# Autodesk Inventor assembly: Ens. Manija
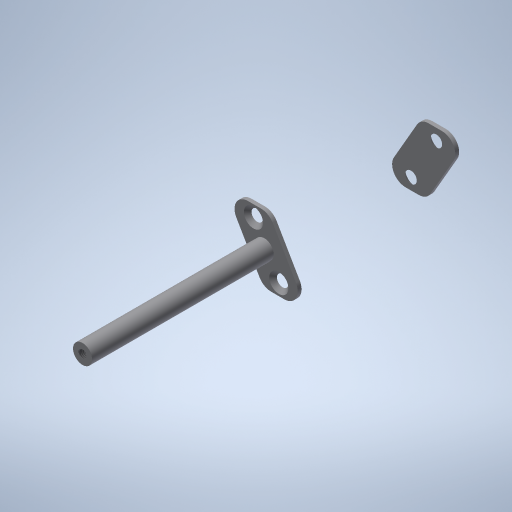
[picture p0: Inventor's stored thumbnail of the model, 512x512]
Saved by Autodesk Inventor 2024.2 (Build 282272000, 272)
## iProperties
Created: 2024-11-25
Part Number: Ens. Manija
Material: Genérico
Document SubType Name: Assembly
Designer: jd.castellanosq
Author: jd.castellanosq
## Documents named in this file (3)
- I:\MICROMECANICA\ALTAS ENERGIAS\Deteccion de Muones\Detectores centelladores\Partes Detectores centelladores\PARTES DC\Manija\Ens. Manija.iam
- I:\MICROMECANICA\ALTAS ENERGIAS\Deteccion de Muones\Detectores centelladores\Partes Detectores centelladores\PARTES DC\Manija\Lamina.ipt
- I:\MICROMECANICA\ALTAS ENERGIAS\Deteccion de Muones\Detectores centelladores\Partes Detectores centelladores\PARTES DC\Manija\eje.ipt
## Components (3 placed, 2 different names)
1. eje:1 — Flush:1, Flush:2, Flush:3, Mate:1
2. Lamina:1
3. Lamina:2
## Relationships (4: Flush 3, Mate 1)
- Flush:1: eje:1
- Flush:2: eje:1
- Flush:3: eje:1
- Mate:1: eje:1
